# Autodesk Inventor assembly: Connessione-D
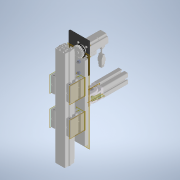
[picture p0: Inventor's stored thumbnail of the model, 180x180]
Saved by Autodesk Inventor 2022 (Build 260153000, 153)
## iProperties
RuleStatus: InUse
Created: 2022-08-22
Part Number: Connessione-D
Document SubType Name: Assembly
Designer: matte
Author: matte
## Documents named in this file (14)
- C:\Users\matte\Documents\GitHub\MDM-CyberOrto-CAD\Dettagli\Connessione-D.iam
- C:\Users\matte\Documents\GitHub\MDM-CyberOrto-CAD\Pezzi singoli\Supporto DX.ipt
- C:\Users\matte\Documents\GitHub\MDM-CyberOrto-CAD\Pezzi singoli\Supporto lineare\Carrello semplice.iam
- C:\Users\matte\Documents\GitHub\MDM-CyberOrto-CAD\Servo Motor 50W\bch2mba531ca5c.ipt
- C:\Users\matte\Documents\GitHub\MDM-CyberOrto-CAD\Trave a terra\Trave a terra.iam
- C:\Users\matte\Documents\GitHub\MDM-CyberOrto-CAD\Parker components\02-Fasteners\16-Screws\01-Metric Screws\01-Button Head\24-120-8.ipt
- C:\Users\matte\Documents\GitHub\MDM-CyberOrto-CAD\Platform.ipt
- C:\Users\matte\Documents\GitHub\MDM-CyberOrto-CAD\Parker components\02-Fasteners\16-Screws\01-Metric Screws\01-Button Head\24-130-6.ipt
- C:\Users\matte\Documents\GitHub\MDM-CyberOrto-CAD\Parker components\02-Fasteners\15-T-Bolts_Nuts_Washers\03-Washers\24-700-6.ipt
- C:\Users\matte\Documents\GitHub\MDM-CyberOrto-CAD\Parker components\02-Fasteners\15-T-Bolts_Nuts_Washers\02-Nuts\24-706-6.ipt
- C:\Users\matte\Documents\GitHub\MDM-CyberOrto-CAD\Inventor Support\Content Center Files\it-IT\ISO 1580\ISO 1580 - M4 x 12_.ipt
- C:\Users\matte\Documents\GitHub\MDM-CyberOrto-CAD\Inventor Support\Content Center Files\it-IT\AS 1474(1)\AS 1474 - M4(1).ipt
- C:\Users\matte\Documents\GitHub\MDM-CyberOrto-CAD\Rack_Pinion\Rack.ipt
- C:\Users\matte\Documents\GitHub\MDM-CyberOrto-CAD\Rack_Pinion\Pinion.ipt
## Components (28 placed, 13 different names)
1. Supporto DX:1
2. Carrello semplice:1 [sub-assembly]
3. 24-120-8:1
4. Platform:1
5. 24-130-6:1
6. 24-700-6:1
7. 24-706-6:1
8. 24-130-6:2
9. 24-700-6:2
10. 24-130-6:3
11. 24-700-6:3
12. 24-130-6:4
13. 24-700-6:4
14. 24-706-6:2
15. 24-706-6:3
16. 24-706-6:4
17. bch2mba531ca5c:1 — Coincidente:37
18. ISO 1580 M4 x 12:1
19. AS 1474 - Metrico M4:1
20. ISO 1580 M4 x 12:2
21. AS 1474 - Metrico M4:2
22. AS 1474 - Metrico M4:3
23. AS 1474 - Metrico M4:4
24. ISO 1580 M4 x 12:3
25. ISO 1580 M4 x 12:4
26. Trave a terra:1 [sub-assembly] — Coincidente:36, Allineato:5
27. Rack:1 — Coincidente:36, Allineato:5
28. Pinion:1 — Coincidente:37
## Relationships (51: Mate 35, Insert 8, Flush 5, Angle 3)
- [Mate]: Supporto DX:1 ↔ Carrello semplice:1
- [Flush]: Supporto DX:1 ↔ Carrello semplice:1
- [Flush]: Supporto DX:1 ↔ Carrello semplice:1
- [Mate]: Carrello semplice:1 ↔ 24-120-8:1
- [Mate]: Carrello semplice:1 ↔ 24-120-8:1
- [Mate]: Carrello semplice:1 ↔ Platform:1
- [Flush]: Carrello semplice:1 ↔ Platform:1
- [Mate]: Carrello semplice:1 ↔ Platform:1
- [Insert]: 24-130-6:1 ↔ 24-700-6:1
- [Insert]: 24-130-6:2 ↔ 24-700-6:2
- [Insert]: 24-130-6:3 ↔ 24-700-6:3
- [Insert]: 24-130-6:4 ↔ 24-700-6:4
- [Insert]: Platform:1 ↔ 24-700-6:4
- [Insert]: Platform:1 ↔ 24-700-6:3
- [Insert]: Platform:1 ↔ 24-700-6:1
- [Insert]: Platform:1 ↔ 24-700-6:2
- [Mate]: 24-706-6:1 ↔ 24-130-6:4
- [Mate]: Carrello semplice:1 ↔ 24-706-6:1
- [Mate]: 24-130-6:3 ↔ 24-706-6:2
- [Mate]: Carrello semplice:1 ↔ 24-706-6:2
- [Mate]: 24-130-6:2 ↔ 24-706-6:4
- [Mate]: Carrello semplice:1 ↔ 24-706-6:4
- [Mate]: 24-130-6:1 ↔ 24-706-6:3
- [Mate]: Carrello semplice:1 ↔ 24-706-6:3
- [Mate]: Platform:1 ↔ bch2mba531ca5c:1
- [Mate]: Platform:1 ↔ bch2mba531ca5c:1
- [Mate]: Platform:1 ↔ bch2mba531ca5c:1
- [Mate]: Platform:1 ↔ ISO 1580 M4 x 12:1
- [Mate]: bch2mba531ca5c:1 ↔ ISO 1580 M4 x 12:1
- [Mate]: ISO 1580 M4 x 12:1 ↔ AS 1474 - Metrico M4:1
- [Mate]: Platform:1 ↔ AS 1474 - Metrico M4:1
- [Mate]: bch2mba531ca5c:1 ↔ ISO 1580 M4 x 12:4
- [Mate]: bch2mba531ca5c:1 ↔ ISO 1580 M4 x 12:4
- [Mate]: AS 1474 - Metrico M4:2 ↔ ISO 1580 M4 x 12:4
- [Mate]: Platform:1 ↔ AS 1474 - Metrico M4:2
- [Mate]: bch2mba531ca5c:1 ↔ ISO 1580 M4 x 12:3
- [Mate]: bch2mba531ca5c:1 ↔ ISO 1580 M4 x 12:3
- [Mate]: AS 1474 - Metrico M4:3 ↔ ISO 1580 M4 x 12:3
- [Mate]: Platform:1 ↔ AS 1474 - Metrico M4:3
- [Mate]: bch2mba531ca5c:1 ↔ ISO 1580 M4 x 12:2
- [Mate]: bch2mba531ca5c:1 ↔ ISO 1580 M4 x 12:2
- [Mate]: ISO 1580 M4 x 12:2 ↔ AS 1474 - Metrico M4:4
- [Mate]: Platform:1 ↔ AS 1474 - Metrico M4:4
- [Angle] (0 deg): Carrello semplice:1 ↔ Trave a terra:1
- [Angle] (0 deg): Carrello semplice:1 ↔ Trave a terra:1
- [Angle] (0 deg): Carrello semplice:1 ↔ Trave a terra:1
- [Flush] (19 mm): Carrello semplice:1 ↔ Trave a terra:1
- [Mate] (20 mm): Carrello semplice:1 ↔ Trave a terra:1
- Coincidente:36 [Mate]: Trave a terra:1 ↔ Rack:1
- Coincidente:37 [Mate]: bch2mba531ca5c:1 ↔ Pinion:1
- Allineato:5 [Flush]: Trave a terra:1 ↔ Rack:1
## Named parameters: d116_d115 = 0 mm, d117_d115 = 0 mm, d118_d115 = 0 mm
